# Autodesk Inventor assembly: Entire Robot assembly
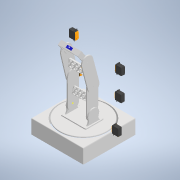
[picture p0: Inventor's stored thumbnail of the model, 180x180]
Saved by Autodesk Inventor 2020.2 (Build 242310000, 310)
## iProperties
Created: 2020-03-31
Part Number: Entire Robot assembly
Document SubType Name: Assembly
Designer: Amaan Khalid
Author: Amaan Khalid
## Documents named in this file (12)
- C:\Users\Amaan Khalid\Desktop\Robotic Arm project\My parts\Entire Robot assembly.iam
- C:\Users\Amaan Khalid\Desktop\Robotic Arm project\My parts\Base Hinge 2x.ipt
- C:\Users\Amaan Khalid\Desktop\Robotic Arm project\My parts\Base Bracket 1x.ipt
- C:\Users\Amaan Khalid\Desktop\Robotic Arm project\My parts\Second Arm.ipt
- C:\Users\Amaan Khalid\Desktop\Robotic Arm project\My parts\Arm support.ipt
- C:\Users\Amaan Khalid\Desktop\Robotic Arm project\My parts\Arm support for bottom arms.ipt
- C:\Users\Amaan Khalid\Desktop\Robotic Arm project\My parts\Rotating Base.ipt
- C:\Users\Amaan Khalid\Desktop\Robotic Arm project\My parts\Base box.ipt
- C:\Users\Amaan Khalid\Desktop\Robotic Arm project\My parts\1st Servo Holder.ipt
- C:\Users\Amaan Khalid\Desktop\Robotic Arm project\My parts\Components Cads\SG90.ipt
- C:\Users\Amaan Khalid\Desktop\Robotic Arm project\My parts\Components Cads\28BYJ-48 stepper motor.iam
- C:\Users\Amaan Khalid\Desktop\Robotic Arm project\My parts\Components Cads\MG996R Servo.ipt
## Components (20 placed, 11 different names)
1. Base Hinge 2x:1 — Mate:2, Rotational:3
2. Base Hinge 2x:2 — Mate:1, Rotational:2
3. Base Bracket 1x:1 — Mate:1, Mate:2, Mate:7, Mate:8, Mate:9
4. Second Arm:2 — Rotational:2, Rotational:4, Mate:4
5. Second Arm:3 — Rotational:3, Rotational:5, Mate:3
6. Second Arm:4 — Rotational:4, Mate:10, Rotational:7
7. Second Arm:5 — Rotational:5, Mate:11
8. Arm support for bottom arms:1 — Mate:3, Mate:4
9. Rotating Base:5 — Mate:7, Mate:8, Mate:9, Rotational:6, Mate:14
10. Base box:1 — Rotational:6
11. Arm support:2 — Mate:10, Mate:11
12. 1st Servo Holder:1 — Rotational:7, Mate:12, Mate:13
13. SG90:2 — Mate:12, Mate:13
14. 28BYJ-48 stepper motor:2 [sub-assembly] — Mate:14
15. MG996R Servo:14
16. MG996R Servo:15
17. MG996R Servo:16
18. MG996R Servo:17
19. MG996R Servo:18
20. MG996R Servo:19
## Relationships (18: Mate 12, RevoluteJoint 6)
- Mate:1: Base Hinge 2x:2 ↔ Base Bracket 1x:1
- Mate:2: Base Hinge 2x:1 ↔ Base Bracket 1x:1
- Rotational:2 [RevoluteJoint]: Base Hinge 2x:2 ↔ Second Arm:2
- Rotational:3 [RevoluteJoint]: Base Hinge 2x:1 ↔ Second Arm:3
- Rotational:4 [RevoluteJoint]: Second Arm:2 ↔ Second Arm:4
- Rotational:5 [RevoluteJoint]: Second Arm:3 ↔ Second Arm:5
- Mate:3: Second Arm:3 ↔ Arm support for bottom arms:1
- Mate:4: Second Arm:2 ↔ Arm support for bottom arms:1
- Mate:7: Base Bracket 1x:1 ↔ Rotating Base:5
- Mate:8: Base Bracket 1x:1 ↔ Rotating Base:5
- Mate:9: Base Bracket 1x:1 ↔ Rotating Base:5
- Mate:10: Second Arm:4 ↔ Arm support:2
- Mate:11: Second Arm:5 ↔ Arm support:2
- Rotational:6 [RevoluteJoint]: Rotating Base:5 ↔ Base box:1
- Rotational:7 [RevoluteJoint]: Second Arm:4 ↔ 1st Servo Holder:1
- Mate:12: 1st Servo Holder:1 ↔ SG90:2
- Mate:13: 1st Servo Holder:1 ↔ SG90:2
- Mate:14: Rotating Base:5 ↔ 28BYJ-48 stepper motor:2
